# Autodesk Inventor assembly: task_hunter
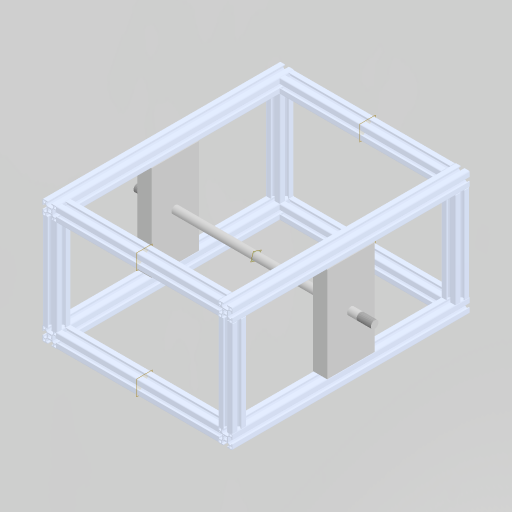
[picture p0: Inventor's stored thumbnail of the model, 512x512]
Saved by Autodesk Inventor 2024 (Build 280153000, 153)
## iProperties
Created: 2024-11-01
Part Number: task_hunter
Document SubType Name: Assembly
Designer: Wicek
Author: Wicek
## Documents named in this file (6)
- C:\Users\fkoba.i_ekonomik\Desktop\Model 3D\task_hunter.iam
- C:\Users\fkoba.i_ekonomik\Desktop\Model 3D\Rama_bok.ipt
- C:\Users\fkoba.i_ekonomik\Desktop\Model 3D\Rama_przód.ipt
- C:\Users\fkoba.i_ekonomik\Desktop\Model 3D\Rama_słupek.ipt
- C:\Users\fkoba.i_ekonomik\Desktop\Model 3D\mocowanie osi.ipt
- C:\Users\fkoba.i_ekonomik\Desktop\Model 3D\oś.ipt
## Components (15 placed, 5 different names)
1. Rama_bok:1 — Zestawiające:3, Równoległe:2, Zestawiające:4, Zestawiające:12, Równoległe:16, Równoległe:17
2. Rama_bok:2 — Równoległe:3, Zestawiające:5, Zestawiające:6, Zestawiające:7, Zestawiające:8, Zestawiające:11, Równoległe:14, Równoległe:5, Równoległe:20
3. Rama_przód:1 — Zestawiające:1, Zestawiające:2, Równoległe:1, Zestawiające:3, Równoległe:2, Zestawiające:4, Równoległe:3, Zestawiające:5, Zestawiające:6, Zestawiające:9, Równoległe:18, Równoległe:19
4. Rama_przód:2 — Zestawiające:7, Zestawiające:8, Zestawiające:10, Równoległe:4, Równoległe:5, Równoległe:15
5. Rama_słupek:1 — Zestawiające:9, Równoległe:19, Równoległe:20
6. Rama_słupek:2 — Zestawiające:12, Równoległe:17, Równoległe:18, Zestawiające:18, Równoległe:25, Równoległe:26, Zestawiające:20
7. Rama_słupek:3 — Zestawiające:11, Równoległe:14, Równoległe:4
8. Rama_słupek:4 — Zestawiające:10, Równoległe:15, Równoległe:16
9. Rama_przód:3 — Zestawiające:13, Zestawiające:14, Równoległe:21
10. Rama_przód:4 — Zestawiające:15, Zestawiające:16, Równoległe:22, Równoległe:23, Równoległe:24, Zestawiające:17, Zestawiające:24
11. Rama_bok:3 — Zestawiające:13, Zestawiające:14, Równoległe:21, Zestawiające:15, Zestawiające:16, Równoległe:22, Zestawiające:21, Równoległe:28
12. Rama_bok:4 — Równoległe:23, Równoległe:24, Zestawiające:17, Zestawiające:18, Równoległe:25, Równoległe:26, Zestawiające:19, Równoległe:27
13. mocowanie osi:1 — Zestawiające:21, Równoległe:28, Zestawiające:22, Zestawiające:23
14. mocowanie osi:2 — Zestawiające:19, Równoległe:27, Zestawiające:20, Zestawiające:22
15. oś:1 — Zestawiające:23, Zestawiające:24
## Relationships (44: Mate 24, Flush 20)
- Zestawiające:1 [Mate]: Rama_przód:1
- Zestawiające:2 [Mate]: Rama_przód:1
- Równoległe:1 [Flush]: Rama_przód:1
- Zestawiające:3 [Mate]: Rama_bok:1 ↔ Rama_przód:1
- Równoległe:2 [Flush]: Rama_bok:1 ↔ Rama_przód:1
- Zestawiające:4 [Mate]: Rama_bok:1 ↔ Rama_przód:1
- Równoległe:3 [Flush]: Rama_bok:2 ↔ Rama_przód:1
- Zestawiające:5 [Mate]: Rama_bok:2 ↔ Rama_przód:1
- Zestawiające:6 [Mate]: Rama_bok:2 ↔ Rama_przód:1
- Zestawiające:7 [Mate]: Rama_bok:2 ↔ Rama_przód:2
- Zestawiające:8 [Mate]: Rama_bok:2 ↔ Rama_przód:2
- Zestawiające:9 [Mate]: Rama_przód:1 ↔ Rama_słupek:1
- Zestawiające:10 [Mate]: Rama_przód:2 ↔ Rama_słupek:4
- Zestawiające:11 [Mate]: Rama_bok:2 ↔ Rama_słupek:3
- Zestawiające:12 [Mate]: Rama_bok:1 ↔ Rama_słupek:2
- Równoległe:14 [Flush]: Rama_bok:2 ↔ Rama_słupek:3
- Równoległe:4 [Flush]: Rama_przód:2 ↔ Rama_słupek:3
- Równoległe:5 [Flush]: Rama_bok:2 ↔ Rama_przód:2
- Równoległe:15 [Flush]: Rama_przód:2 ↔ Rama_słupek:4
- Równoległe:16 [Flush]: Rama_bok:1 ↔ Rama_słupek:4
- Równoległe:17 [Flush]: Rama_bok:1 ↔ Rama_słupek:2
- Równoległe:18 [Flush]: Rama_przód:1 ↔ Rama_słupek:2
- Równoległe:19 [Flush]: Rama_przód:1 ↔ Rama_słupek:1
- Równoległe:20 [Flush]: Rama_bok:2 ↔ Rama_słupek:1
- Zestawiające:13 [Mate]: Rama_przód:3 ↔ Rama_bok:3
- Zestawiające:14 [Mate]: Rama_przód:3 ↔ Rama_bok:3
- Równoległe:21 [Flush]: Rama_przód:3 ↔ Rama_bok:3
- Zestawiające:15 [Mate]: Rama_przód:4 ↔ Rama_bok:3
- Zestawiające:16 [Mate]: Rama_przód:4 ↔ Rama_bok:3
- Równoległe:22 [Flush]: Rama_przód:4 ↔ Rama_bok:3
- Równoległe:23 [Flush]: Rama_przód:4 ↔ Rama_bok:4
- Równoległe:24 [Flush]: Rama_przód:4 ↔ Rama_bok:4
- Zestawiające:17 [Mate]: Rama_przód:4 ↔ Rama_bok:4
- Zestawiające:18 [Mate]: Rama_słupek:2 ↔ Rama_bok:4
- Równoległe:25 [Flush]: Rama_słupek:2 ↔ Rama_bok:4
- Równoległe:26 [Flush]: Rama_słupek:2 ↔ Rama_bok:4
- Zestawiające:19 [Mate]: Rama_bok:4 ↔ mocowanie osi:2
- Równoległe:27 [Flush]: Rama_bok:4 ↔ mocowanie osi:2
- Zestawiające:20 [Mate] (220 mm): Rama_słupek:2 ↔ mocowanie osi:2
- Zestawiające:21 [Mate]: Rama_bok:3 ↔ mocowanie osi:1
- Równoległe:28 [Flush]: Rama_bok:3 ↔ mocowanie osi:1
- Zestawiające:22 [Mate]: mocowanie osi:1 ↔ mocowanie osi:2
- Zestawiające:23 [Mate]: mocowanie osi:1 ↔ oś:1
- Zestawiające:24 [Mate]: Rama_przód:4 ↔ oś:1
